# Autodesk Inventor assembly: flat 0.125A
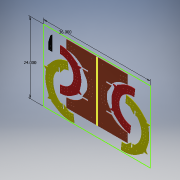
[picture p0: Inventor's stored thumbnail of the model, 180x180]
Saved by Autodesk Inventor 2016 (Build 200138000, 138)
## iProperties
Created: 2016-02-06
Part Number: flat 0.125A
Document SubType Name: Assembly
Designer: Scott
Author: Scott
## Documents named in this file (5)
- F:\Dropbox\CubeSat\Cleaned_Up_Helmholtz_Model_for_Manual\Flat_Patterns\flat 0.125A.iam
- F:\Dropbox\CubeSat\Cleaned_Up_Helmholtz_Model_for_Manual\Parts\Small_Coil_Outer.ipt
- F:\Dropbox\CubeSat\Cleaned_Up_Helmholtz_Model_for_Manual\Parts\Medium_Coil_Outer.ipt
- F:\Dropbox\CubeSat\Cleaned_Up_Helmholtz_Model_for_Manual\Parts\Large_Coil_Outer_Bottom.ipt
- F:\Dropbox\CubeSat\Cleaned_Up_Helmholtz_Model_for_Manual\Parts\Coil_Retainer_2_Hole.ipt
## Components (7 placed, 4 different names)
1. Large_Coil_Outer_Bottom:1 — Flush:21, Mate:1
2. Large_Coil_Outer_Bottom:2 — Flush:21, Mate:1, Flush:22
3. Medium_Coil_Outer:3 — Flush:20
4. Medium_Coil_Outer:4
5. Small_Coil_Outer:1 — Flush:20
6. Small_Coil_Outer:4
7. Coil_Retainer_2_Hole:1 — Flush:22
## Relationships (4: Flush 3, Mate 1)
- Flush:20: Medium_Coil_Outer:3 ↔ Small_Coil_Outer:1
- Flush:21: Large_Coil_Outer_Bottom:1 ↔ Large_Coil_Outer_Bottom:2
- Mate:1 (12.7 mm): Large_Coil_Outer_Bottom:1 ↔ Large_Coil_Outer_Bottom:2
- Flush:22: Large_Coil_Outer_Bottom:2 ↔ Coil_Retainer_2_Hole:1
